# Autodesk Inventor assembly: afscherming
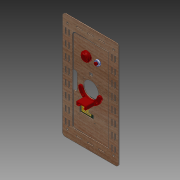
[picture p0: Inventor's stored thumbnail of the model, 180x180]
Saved by Autodesk Inventor 2015 (Build 190159000, 159)
## iProperties
Created: 2015-12-31
Part Number: afscherming
Document SubType Name: Assembly
Designer: david
Author: david
## Documents named in this file (7)
- Z:\gip\Inventor\generatie 7\Frame\afscherming.iam
- Z:\gip\Inventor\generatie 7\Frame\doos\prim.ipt
- Z:\gip\Inventor\generatie 7\Frame\doos\binnenplaat.ipt
- Z:\gip\Inventor\generatie 7\Frame\Electronica\raspberry pi\raspberry pi.iam
- Z:\gip\Inventor\generatie 7\Frame\doos\Buton_1.ipt
- Z:\gip\Inventor\generatie 7\Frame\doos\Button2.iam
- Z:\gip\Inventor\generatie 7\Camerahouder.ipt
## Components (6 placed, 6 different names)
1. prim:1 — Mate:1, Mate:2
2. binnenplaat:1 — Mate:1, Mate:2, Mate:3, Mate:4, Mate:5, Mate:6, Mate:7, Mate:8, Mate:9, Flush:1
3. raspberry pi:1 [sub-assembly] — Mate:3, Mate:4, Mate:5
4. Buton_1:1 — Mate:6, Mate:7
5. Button2:1 [sub-assembly] — Mate:8, Mate:9
6. Camerahouder:1 — Flush:1
## Relationships (10: Mate 9, Flush 1)
- Mate:1: prim:1 ↔ binnenplaat:1
- Mate:2 (2.5 mm): prim:1 ↔ binnenplaat:1
- Mate:3: binnenplaat:1 ↔ raspberry pi:1
- Mate:4 (5 mm): binnenplaat:1 ↔ raspberry pi:1
- Mate:5: binnenplaat:1 ↔ raspberry pi:1
- Mate:6: binnenplaat:1 ↔ Buton_1:1
- Mate:7: binnenplaat:1 ↔ Buton_1:1
- Mate:8: binnenplaat:1 ↔ Button2:1
- Mate:9: binnenplaat:1 ↔ Button2:1
- Flush:1: binnenplaat:1 ↔ Camerahouder:1
